# Autodesk Inventor assembly: Zespół1
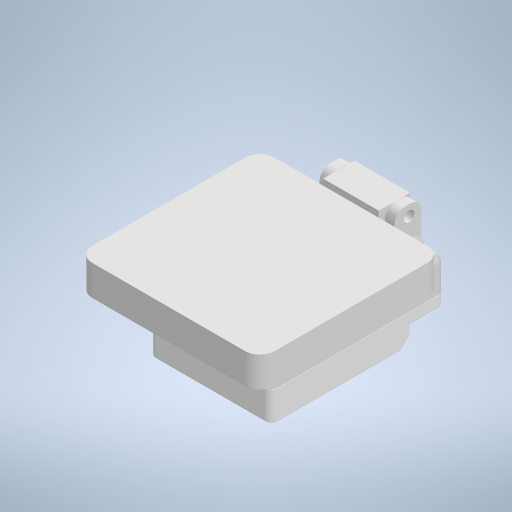
[picture p0: Inventor's stored thumbnail of the model, 512x512]
Saved by Autodesk Inventor 2024 (Build 280153000, 153)
## iProperties
Created: 2023-12-07
Part Number: Zespół1
Document SubType Name: Assembly
Designer: pient
Author: pient
## Documents named in this file (4)
- C:\Users\pient\Desktop\lampa\Zespół1.iam
- C:\Users\pient\Desktop\lampa\gura.ipt
- C:\Users\pient\Desktop\lampa\lampa.ipt
- C:\Users\pient\Desktop\lampa\batteryLamp-main_bottom.ipt
## Components (3 placed, 3 different names)
1. gura:1 — Obrotowe:1, Sztywne:1
2. lampa:2 — Obrotowe:1
3. batteryLamp-main_bottom:1 — Sztywne:1
## Relationships (2: RevoluteJoint 1, WeldJoint 1)
- Obrotowe:1 [RevoluteJoint]: gura:1 ↔ lampa:2
- Sztywne:1 [WeldJoint] (0.2 mm): gura:1 ↔ batteryLamp-main_bottom:1
